# Autodesk Inventor assembly: OBG-Akkuabdeckung
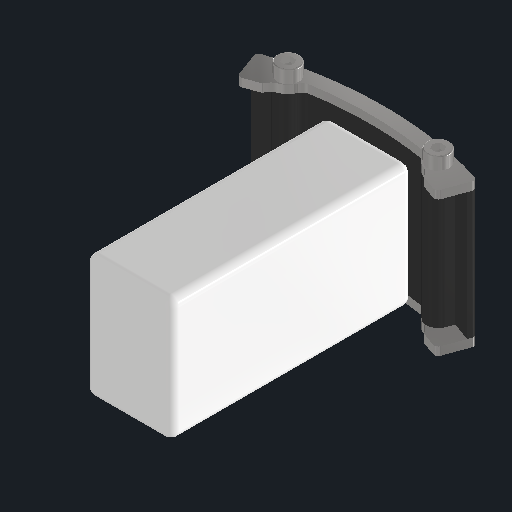
[picture p0: Inventor's stored thumbnail of the model, 512x512]
Saved by Autodesk Inventor 2025.2 (Build 292293000, 293)
## iProperties
Created: 2025-03-27
Part Number: OBG-Akkuabdeckung
Document SubType Name: Assembly
Designer: Faabs
Author: Faabs
## Documents named in this file (5)
- C:\Users\Faabs\Desktop\TeamFaabs-CAD v2023\OBG\Akku\OBG-Akkuabdeckung.iam
- C:\Users\Faabs\Desktop\TeamFaabs-CAD v2023\OBG\Akku\Akkuabdeckung.ipt
- C:\Users\Faabs\Desktop\TeamFaabs-CAD v2023\OBG\Akku\Schutzring_Akku.ipt
- C:\Users\Faabs\Desktop\TeamFaabs-CAD v2023\Verbindungselemente\DIN 912\DIN 912 - M3 x 0,5 x 30 x 18.ipt
- C:\Users\Faabs\Desktop\TeamFaabs-CAD v2023\OBG\Akku\12V Akku.ipt
## Components (6 placed, 4 different names)
1. Akkuabdeckung:1 — Passend:1, Passend:2, Passend:3, Passend:4, Passend:5, Passend:6, Passend:7, Passend:8, Passend:9, Tangential:1
2. Schutzring_Akku:1 — Passend:1, Passend:5, Passend:9, Einfügen:1, Einfügen:2
3. Schutzring_Akku:2 — Passend:6, Passend:7, Passend:8, Fluchtend:1
4. DIN 912 - ersetzt durch DIN EN ISO 4762 M3 x 30:1 — Einfügen:1
5. DIN 912 - ersetzt durch DIN EN ISO 4762 M3 x 30:2 — Einfügen:2
6. 12V Akku:1 — Fluchtend:1, Passend:10, Tangential:1
## Relationships (14: Mate 10, Insert 2, Flush 1, Tangent 1)
- Passend:1 [Mate]: Akkuabdeckung:1 ↔ Schutzring_Akku:1
- Passend:2 [Mate]: Akkuabdeckung:1
- Passend:3 [Mate]: Akkuabdeckung:1
- Passend:4 [Mate]: Akkuabdeckung:1
- Passend:5 [Mate]: Akkuabdeckung:1 ↔ Schutzring_Akku:1
- Passend:6 [Mate]: Akkuabdeckung:1 ↔ Schutzring_Akku:2
- Passend:7 [Mate]: Akkuabdeckung:1 ↔ Schutzring_Akku:2
- Passend:8 [Mate]: Akkuabdeckung:1 ↔ Schutzring_Akku:2
- Passend:9 [Mate]: Akkuabdeckung:1 ↔ Schutzring_Akku:1
- Einfügen:1 [Insert]: Schutzring_Akku:1 ↔ DIN 912 - ersetzt durch DIN EN ISO 4762 M3 x 30:1
- Einfügen:2 [Insert]: Schutzring_Akku:1 ↔ DIN 912 - ersetzt durch DIN EN ISO 4762 M3 x 30:2
- Fluchtend:1 [Flush]: Schutzring_Akku:2 ↔ 12V Akku:1
- Passend:10 [Mate]: 12V Akku:1
- Tangential:1: Akkuabdeckung:1 ↔ 12V Akku:1
